# Autodesk Inventor assembly: Motor + sprocket + translock
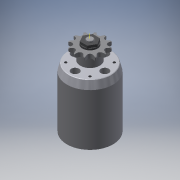
[picture p0: Inventor's stored thumbnail of the model, 180x180]
Saved by Autodesk Inventor 2018 (Build 220112000, 112)
## iProperties
Created: 2018-08-13
Part Number: Motor + sprocket + translock
Document SubType Name: Assembly
Designer: ruben
Author: ruben
## Documents named in this file (4)
- C:\Users\ruben\Documents\Inventor\Electric-Scooter\Transmission\Motor + sprocket + translock.iam
- C:\Users\ruben\Documents\Inventor\Electric-Scooter\Transmission\Sprocket 3-8x7-32 12T.ipt
- C:\Users\ruben\Documents\Inventor\Electric-Scooter\Transmission\Translock taperlock.ipt
- C:\Users\ruben\Documents\Inventor\Electric-Scooter\Transmission\Turnigy Brushless DC Motor.ipt
## Components (3 placed, 3 different names)
1. Sprocket 3-8x7-32 12T:1 — Insert:2
2. Translock taperlock:1 — Insert:1
3. Turnigy Brushless DC Motor:1 — Insert:1, Insert:2, Mate:1
## Relationships (3: Insert 2, Mate 1)
- Insert:1 (1 mm): Translock taperlock:1 ↔ Turnigy Brushless DC Motor:1
- Insert:2 (-6 mm): Sprocket 3-8x7-32 12T:1 ↔ Turnigy Brushless DC Motor:1
- Mate:1: Turnigy Brushless DC Motor:1
